# Autodesk Inventor assembly: IG42C-39.2Dtype _1_
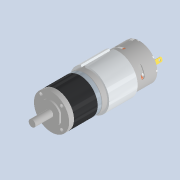
[picture p0: Inventor's stored thumbnail of the model, 180x180]
Saved by Autodesk Inventor 2021 (Build 250183000, 183)
## iProperties
Created: 2020-02-10
Part Number: IG42C-39.2Dtype _1_
Document SubType Name: Assembly
Designer: Hagihara Yuya
Mass: 551 g
Surface Area: 616.919 cm^2
Volume: 70.3897 cm^3
Author: Hagihara Yuya
Revision Number: NONE
## Documents named in this file (6)
- C:\Users\Hagihara Yuya\Documents\GrabCAD\NHK2021\BasicParts\よく使う部品（萩原）\Motor\775\Geared775.iam
- C:\Users\Hagihara Yuya\Documents\GrabCAD\NHK2021\BasicParts\よく使う部品（萩原）\Motor\775\フランジ.ipt
- C:\Users\Hagihara Yuya\Documents\GrabCAD\NHK2021\BasicParts\よく使う部品（萩原）\Motor\775\39.2.ipt
- C:\Users\Hagihara Yuya\Documents\GrabCAD\NHK2021\BasicParts\よく使う部品（萩原）\Motor\775\フロントカバー.ipt
- C:\Users\Hagihara Yuya\Documents\GrabCAD\NHK2021\BasicParts\よく使う部品（萩原）\Motor\775\Dカットシャフト.ipt
- C:\Users\Hagihara Yuya\Documents\GrabCAD\NHK2021\BasicParts\よく使う部品（萩原）\Motor\775\775.iam
## Components (5 placed, 5 different names)
1. NAUO1 — リジッド:1
2. NAUO2
3. NAUO3
4. NAUO4
5. 775:1 [sub-assembly] — リジッド:1
## Relationships (1: WeldJoint 1)
- リジッド:1 [WeldJoint]: NAUO1 ↔ 775:1
